# Autodesk Inventor assembly: Supershifter Hex Shaft Standard subassembly
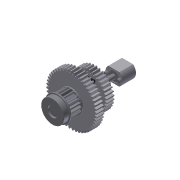
[picture p0: Inventor's stored thumbnail of the model, 180x180]
Saved by Autodesk Inventor 2011 (Build 150239000, 239)
## iProperties
Created: 2011-07-04
Part Number: Supershifter Hex Shaft Standard subassembly
Document SubType Name: Assembly
Designer: Dan Niemitalo
Author: Dan Niemitalo
## Documents named in this file (12)
- H:\Nemo\Documents\Robotics\COTS Parts\Gearboxes\Shafts\Supershifter Hex Shaft Standard subassembly.iam
- H:\Nemo\Documents\Robotics\COTS Parts\Gearboxes\Shifters\Roll Pin 925x100.ipt
- H:\Nemo\Documents\Robotics\COTS Parts\Gearboxes\Shafts\Supershifter Hex Shaft.ipt
- H:\Nemo\Documents\Robotics\COTS Parts\Gearboxes\Bearings\Bearing FR6zz.ipt
- H:\Nemo\Documents\Robotics\COTS Parts\Gearboxes\Bearings\Bearing FR6.ipt
- H:\Nemo\Documents\Robotics\COTS Parts\Gearboxes\Bearings\Bearing FR8zz.ipt
- H:\Nemo\Documents\Robotics\COTS Parts\Gearboxes\Bearings\Bearing R8.ipt
- H:\Nemo\Documents\Robotics\COTS Parts\Gearboxes\Shifters\Dog Gear.ipt
- H:\Nemo\Documents\Robotics\COTS Parts\Gearboxes\Gears\Gear 20dp 500key 20T.ipt
- H:\Nemo\Documents\Robotics\COTS Parts\Gearboxes\Gears\Gear 20dp 1125dog 48T.ipt
- H:\Nemo\Documents\Robotics\COTS Parts\Gearboxes\Gears\Gear 20dp 875dog 35T.ipt
- H:\Nemo\Documents\Robotics\COTS Parts\Gearboxes\Shifters\Shift Block subassembly.iam
## Components (11 placed, 11 different names)
1. Bearing FR8zz:1 — Mate:19, Mate:22
2. Bearing FR6zz:1 — Mate:22
3. Bearing FR6:1 — Insert:4, Insert:5
4. Supershifter Hex Shaft — Mate:6, Mate:7, Mate:16, Angle:1, Mate:17, Insert:5, Mate:20
5. Bearing R8:1 — Insert:3, Mate:17, Mate:18
6. Dog gear — Mate:6, Mate:7, Mate:15, Flush:2
7. Roll Pin 925x100:1 — Mate:15, Flush:2, Mate:21
8. Gear 20T 20dp 500key:1 — Mate:16, Angle:1, Mate:18, Mate:19
9. Gear 48T dog shift:1 — Insert:3
10. Gear 35T dog shift:1 — Insert:4
11. Shift Block subassembly:1 [sub-assembly] — Mate:20, Mate:21
## Relationships (17: Mate 11, Insert 4, Flush 1, Angle 1)
- [Mate]: Bearing FR8zz:1 ↔ Supershifter Hex Shaft
- [Insert]: Bearing FR6zz:1 ↔ Bearing FR6:1
- Mate:6: Supershifter Hex Shaft ↔ Dog gear
- Mate:7: Supershifter Hex Shaft ↔ Dog gear
- Mate:15: Dog gear ↔ Roll Pin 925x100:1
- Flush:2: Dog gear ↔ Roll Pin 925x100:1
- Mate:16: Supershifter Hex Shaft ↔ Gear 20T 20dp 500key:1
- Angle:1 (0 deg): Supershifter Hex Shaft ↔ Gear 20T 20dp 500key:1
- Insert:3: Bearing R8:1 ↔ Gear 48T dog shift:1
- Mate:17: Supershifter Hex Shaft ↔ Bearing R8:1
- Insert:4: Bearing FR6:1 ↔ Gear 35T dog shift:1
- Insert:5: Bearing FR6:1 ↔ Supershifter Hex Shaft
- Mate:18: Bearing R8:1 ↔ Gear 20T 20dp 500key:1
- Mate:19: Bearing FR8zz:1 ↔ Gear 20T 20dp 500key:1
- Mate:20: Supershifter Hex Shaft ↔ Shift Block subassembly:1
- Mate:21: Roll Pin 925x100:1 ↔ Shift Block subassembly:1
- Mate:22 (-50.8 mm): Bearing FR8zz:1 ↔ Bearing FR6zz:1
